# Autodesk Inventor assembly: stay
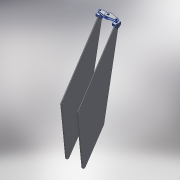
[picture p0: Inventor's stored thumbnail of the model, 180x180]
Saved by Autodesk Inventor 2018.2 (Build 222227000, 227)
## iProperties
Created: 2017-12-11
Part Number: stay
Material: 一般
Document SubType Name: Assembly
Designer: kuwano
Mass: 37579.8 g
Surface Area: 48667.5 cm^2
Volume: 32484 cm^3
Density: 1.15687 g/cm^3
Author: kuwano
## Documents named in this file (3)
- D:\kuwano\Documents\Inventor\KITformula\AeroCAD2018\CAD\Inventor\製作用CAD\R-wing\parts\stay.iam
- D:\kuwano\Documents\Inventor\KITformula\AeroCAD2018\CAD\Inventor\製作用CAD\R-wing\parts\swan_plate.ipt
- D:\kuwano\Documents\Inventor\KITformula\AeroCAD2018\CAD\Inventor\製作用CAD\R-wing\parts\joint\joint.iam
## Components (3 placed, 2 different names)
1. swan_plate:1 — メイト:17, フラッシュ:3, フラッシュ:4, フラッシュ:5, メイト:20
2. swan_plate:2 — フラッシュ:3, フラッシュ:4, フラッシュ:5, フラッシュ:22
3. joint:1 [sub-assembly] — メイト:17, 角度:1, メイト:20, フラッシュ:22
## Relationships (7: Flush 4, Mate 2, Angle 1)
- メイト:17 [Mate]: swan_plate:1 ↔ joint:1
- フラッシュ:3 [Flush]: swan_plate:1 ↔ swan_plate:2
- フラッシュ:4 [Flush]: swan_plate:1 ↔ swan_plate:2
- フラッシュ:5 [Flush] (100 mm): swan_plate:1 ↔ swan_plate:2
- 角度:1 [Angle] (0 deg): joint:1
- メイト:20 [Mate]: swan_plate:1 ↔ joint:1
- フラッシュ:22 [Flush]: swan_plate:2 ↔ joint:1
